# Autodesk Inventor assembly: bras
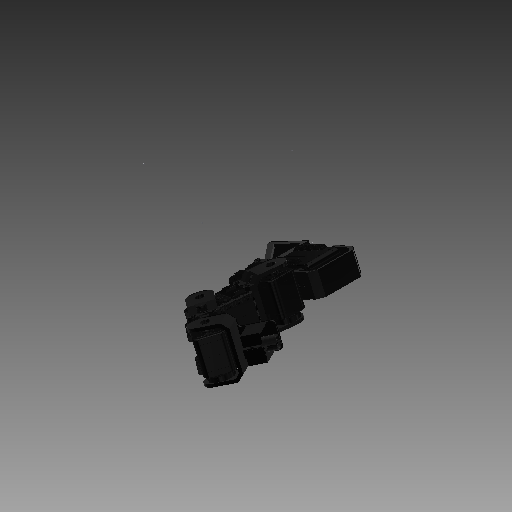
[picture p0: Inventor's stored thumbnail of the model, 512x512]
Saved by Autodesk Inventor 2019 (Build 230136000, 136)
## iProperties
Created: 2019-03-25
Part Number: bras
Document SubType Name: Assembly
Designer: franc
Author: franc
## Documents named in this file (7)
- C:\Users\franc\Desktop\EsialRobotik\Mecanique\2019\robot\bras\bras.iam
- C:\Users\franc\Desktop\EsialRobotik\Mecanique\2019\robot\bras\socleTestBrasVentouse.ipt
- C:\Users\franc\Desktop\EsialRobotik\Mecanique\composants\AX12\AX12.iam
- C:\Users\franc\Desktop\EsialRobotik\Mecanique\2019\robot\bras\axe1BrasVentouse.ipt
- C:\Users\franc\Desktop\EsialRobotik\Mecanique\2019\robot\bras\axe4BrasVentouse.ipt
- C:\Users\franc\Desktop\EsialRobotik\Mecanique\2019\robot\bras\axe2BrasVentouse.ipt
- C:\Users\franc\Desktop\EsialRobotik\Mecanique\2019\robot\bras\supportTestVentouse.ipt
## Components (10 placed, 6 different names)
1. socleTestBrasVentouse:1 — Placage:1, Placage:2, Placage:3
2. AX12:1 [sub-assembly] — Placage:1, Placage:2, Placage:3, Placage:4, Placage:5, Placage:6
3. AX12:2 [sub-assembly] — Placage:7, Placage:8, Placage:9, Placage:10, Placage:11, Placage:12
4. AX12:3 [sub-assembly] — Placage:13, Placage:14, Placage:15, Placage:16, Placage:17, Placage:18
5. AX12:4 [sub-assembly] — Placage:19, Placage:20, Placage:21, Placage:22, Placage:23, Placage:24
6. axe1BrasVentouse:1 — Placage:4, Placage:5, Placage:6, Placage:7, Placage:8, Placage:9
7. axe4BrasVentouse:1 — Placage:10, Placage:11, Placage:12, Placage:13, Placage:14, Placage:15
8. axe4BrasVentouse:2 — Placage:16, Placage:17, Placage:18, Placage:19, Placage:20, Placage:21
9. axe2BrasVentouse:1 — Placage:22, Placage:23, Placage:24, Placage:25, Placage:26, Angle:1
10. supportTestVentouse:1 — Placage:25, Placage:26, Angle:1
## Relationships (27: Mate 26, Angle 1)
- Placage:1 [Mate]: socleTestBrasVentouse:1 ↔ AX12:1
- Placage:2 [Mate]: socleTestBrasVentouse:1 ↔ AX12:1
- Placage:3 [Mate]: socleTestBrasVentouse:1 ↔ AX12:1
- Placage:4 [Mate]: AX12:1 ↔ axe1BrasVentouse:1
- Placage:5 [Mate]: AX12:1 ↔ axe1BrasVentouse:1
- Placage:6 [Mate]: AX12:1 ↔ axe1BrasVentouse:1
- Placage:7 [Mate]: AX12:2 ↔ axe1BrasVentouse:1
- Placage:8 [Mate]: AX12:2 ↔ axe1BrasVentouse:1
- Placage:9 [Mate]: AX12:2 ↔ axe1BrasVentouse:1
- Placage:10 [Mate]: AX12:2 ↔ axe4BrasVentouse:1
- Placage:11 [Mate]: AX12:2 ↔ axe4BrasVentouse:1
- Placage:12 [Mate]: AX12:2 ↔ axe4BrasVentouse:1
- Placage:13 [Mate]: AX12:3 ↔ axe4BrasVentouse:1
- Placage:14 [Mate]: AX12:3 ↔ axe4BrasVentouse:1
- Placage:15 [Mate]: AX12:3 ↔ axe4BrasVentouse:1
- Placage:16 [Mate]: AX12:3 ↔ axe4BrasVentouse:2
- Placage:17 [Mate]: AX12:3 ↔ axe4BrasVentouse:2
- Placage:18 [Mate]: AX12:3 ↔ axe4BrasVentouse:2
- Placage:19 [Mate]: AX12:4 ↔ axe4BrasVentouse:2
- Placage:20 [Mate]: AX12:4 ↔ axe4BrasVentouse:2
- Placage:21 [Mate]: AX12:4 ↔ axe4BrasVentouse:2
- Placage:22 [Mate]: AX12:4 ↔ axe2BrasVentouse:1
- Placage:23 [Mate]: AX12:4 ↔ axe2BrasVentouse:1
- Placage:24 [Mate]: AX12:4 ↔ axe2BrasVentouse:1
- Placage:25 [Mate]: axe2BrasVentouse:1 ↔ supportTestVentouse:1
- Placage:26 [Mate]: axe2BrasVentouse:1 ↔ supportTestVentouse:1
- Angle:1 (180 deg): axe2BrasVentouse:1 ↔ supportTestVentouse:1
